# Autodesk Inventor assembly: Assembly1
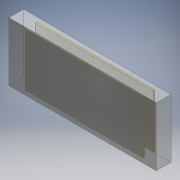
[picture p0: Inventor's stored thumbnail of the model, 180x180]
Saved by Autodesk Inventor 2019.4 (Build 234330000, 330)
## iProperties
Created: 2020-01-02
Part Number: Assembly1
Material: 一般
Document SubType Name: Assembly
Designer: Hideto Niwa
Author: Hideto Niwa
## Documents named in this file (3)
- C:\Users\Hideto Niwa\Desktop\NishikawaLab\卒論\CAD\Assembly1.iam
- C:\Users\Hideto Niwa\Desktop\NishikawaLab\卒論\CAD\導電性布.ipt
- C:\Users\Hideto Niwa\Desktop\NishikawaLab\卒論\CAD\シリコン.ipt
## Components (3 placed, 2 different names)
1. 導電性布:1 — フラッシュ:1, フラッシュ:4, フラッシュ:5
2. 導電性布:2 — フラッシュ:2, フラッシュ:3, フラッシュ:4, フラッシュ:6
3. シリコン:1 — フラッシュ:1, フラッシュ:2, フラッシュ:3, フラッシュ:5, フラッシュ:6
## Relationships (6: Flush 6)
- フラッシュ:1 [Flush] (-5 mm): 導電性布:1 ↔ シリコン:1
- フラッシュ:2 [Flush] (5 mm): 導電性布:2 ↔ シリコン:1
- フラッシュ:3 [Flush] (1 mm): 導電性布:2 ↔ シリコン:1
- フラッシュ:4 [Flush]: 導電性布:1 ↔ 導電性布:2
- フラッシュ:5 [Flush] (0.5 mm): 導電性布:1 ↔ シリコン:1
- フラッシュ:6 [Flush] (-0.5 mm): 導電性布:2 ↔ シリコン:1
